# Autodesk Inventor assembly: EnsamblajeCaja
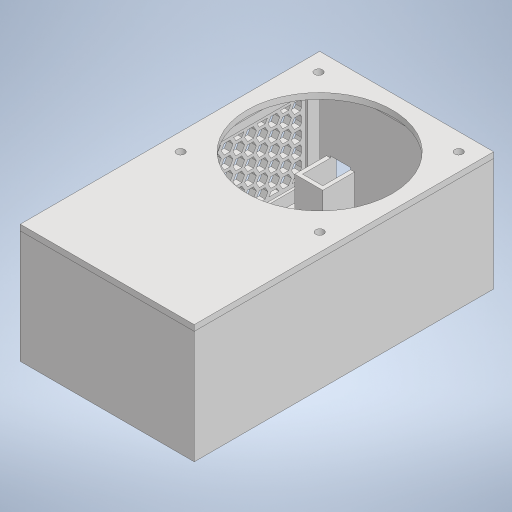
[picture p0: Inventor's stored thumbnail of the model, 512x512]
Saved by Autodesk Inventor 2024 (Build 280153000, 153)
## iProperties
Created: 2023-11-28
Part Number: EnsamblajeCaja
Document SubType Name: Assembly
Designer: sergi
Author: sergi
## Documents named in this file (4)
- C:\Users\sergi\OneDrive\Escritorio\proyectos\3004773_DIY_Dremel_CNC\EnsamblajeCaja.iam
- C:\Users\sergi\OneDrive\Escritorio\proyectos\3004773_DIY_Dremel_CNC\CajaControladora.ipt
- C:\Users\sergi\OneDrive\Escritorio\proyectos\3004773_DIY_Dremel_CNC\Ventilacion.ipt
- C:\Users\sergi\OneDrive\Escritorio\proyectos\3004773_DIY_Dremel_CNC\TapaControladora.ipt
## Components (3 placed, 3 different names)
1. CajaControladora:1 — Coincidencia:1, Coincidencia:2, Coincidencia:3, Coincidencia:4, Coincidencia:5, Coincidencia:6
2. Ventilacion:1 — Coincidencia:1, Coincidencia:2, Coincidencia:3
3. TapaControladora:1 — Coincidencia:4, Coincidencia:5, Coincidencia:6
## Relationships (6: Mate 6)
- Coincidencia:1 [Mate] (0.25 mm): CajaControladora:1 ↔ Ventilacion:1
- Coincidencia:2 [Mate] (0.25 mm): CajaControladora:1 ↔ Ventilacion:1
- Coincidencia:3 [Mate]: CajaControladora:1 ↔ Ventilacion:1
- Coincidencia:4 [Mate]: CajaControladora:1 ↔ TapaControladora:1
- Coincidencia:5 [Mate] (0.25 mm): CajaControladora:1 ↔ TapaControladora:1
- Coincidencia:6 [Mate] (0.25 mm): CajaControladora:1 ↔ TapaControladora:1
